# Autodesk Inventor assembly: USE THIS ball intake design
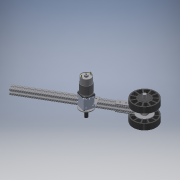
[picture p0: Inventor's stored thumbnail of the model, 180x180]
Saved by Autodesk Inventor 2019 (Build 230136000, 136)
## iProperties
Created: 2019-01-18
Part Number: USE THIS ball intake design
Document SubType Name: Assembly
Designer: s-2513225
Author: s-2513225
## Documents named in this file (9)
- G:\Robotics\Ball Intake 2019\arm assembly left.iam
- G:\Robotics\Ball Intake 2019\wheel tip.ipt
- G:\Robotics\Ball Intake 2019\16in 8020_Shrinkwrap_1.ipt
- G:\Robotics\Ball Intake 2019\0_500_ID_x_1_125_OD_x_0_313_WD_Flanged_Bearing_217-2731.ipt
- G:\Robotics\Ball Intake 2019\motor extension.ipt
- G:\Robotics\Ball Intake 2019\VersaPlanetary_v1_Single_Stage_10_1_with_775_Series.ipt
- G:\Robotics\Ball Intake 2019\am-3480 4IN 500Hex Bore Compliant Wheel.ipt
- G:\Robotics\Ball Intake 2019\hex shaft for wheels.ipt
- G:\Robotics\Ball Intake 2019\wheel spacer.ipt
## Components (12 placed, 8 different names)
1. wheel tip:3 — Mate:14, Mate:34, Flush:9, Flush:10
2. wheel tip:4 — Mate:15, Flush:5, Mate:18, Flush:11
3. 16in 8020_Shrinkwrap_1:1 — Mate:14, Mate:15, Mate:19, Mate:33, Flush:10, Flush:11, Flush:12
4. 0_500_ID_x_1_125_OD_x_0_313_WD_Flanged_Bearing_217-2731:1 — Flush:5, Mate:18, Mate:29
5. 0_500_ID_x_1_125_OD_x_0_313_WD_Flanged_Bearing_217-2731:2 — Mate:34, Flush:9, Mate:35
6. motor extension:1 — Mate:19, Flush:7, Mate:20, Flush:12
7. 0_500_ID_x_1_125_OD_x_0_313_WD_Flanged_Bearing_217-2731:3 — Flush:7, Mate:20, Mate:22, Mate:23
8. VersaPlanetary_v1_Single_Stage_10_1_with_775_Series:1 — Mate:22, Mate:23
9. am-3480 4IN 500Hex Bore Compliant Wheel:1 — Mate:24, Mate:25
10. hex shaft for wheels:1 — Mate:24, Mate:25, Mate:26, Mate:27, Mate:31, Mate:32
11. wheel spacer:1 — Mate:26, Mate:27, Mate:29, Mate:35
12. am-3480 4IN 500Hex Bore Compliant Wheel:2 — Mate:31, Mate:32
## Relationships (23: Mate 17, Flush 6)
- Mate:14: wheel tip:3 ↔ 16in 8020_Shrinkwrap_1:1
- Mate:15: wheel tip:4 ↔ 16in 8020_Shrinkwrap_1:1
- Flush:5: wheel tip:4 ↔ 0_500_ID_x_1_125_OD_x_0_313_WD_Flanged_Bearing_217-2731:1
- Mate:18: wheel tip:4 ↔ 0_500_ID_x_1_125_OD_x_0_313_WD_Flanged_Bearing_217-2731:1
- Mate:19: 16in 8020_Shrinkwrap_1:1 ↔ motor extension:1
- Flush:7: motor extension:1 ↔ 0_500_ID_x_1_125_OD_x_0_313_WD_Flanged_Bearing_217-2731:3
- Mate:20: motor extension:1 ↔ 0_500_ID_x_1_125_OD_x_0_313_WD_Flanged_Bearing_217-2731:3
- Mate:22: 0_500_ID_x_1_125_OD_x_0_313_WD_Flanged_Bearing_217-2731:3 ↔ VersaPlanetary_v1_Single_Stage_10_1_with_775_Series:1
- Mate:23: 0_500_ID_x_1_125_OD_x_0_313_WD_Flanged_Bearing_217-2731:3 ↔ VersaPlanetary_v1_Single_Stage_10_1_with_775_Series:1
- Mate:24: am-3480 4IN 500Hex Bore Compliant Wheel:1 ↔ hex shaft for wheels:1
- Mate:25: am-3480 4IN 500Hex Bore Compliant Wheel:1 ↔ hex shaft for wheels:1
- Mate:26: hex shaft for wheels:1 ↔ wheel spacer:1
- Mate:27: hex shaft for wheels:1 ↔ wheel spacer:1
- Mate:29: 0_500_ID_x_1_125_OD_x_0_313_WD_Flanged_Bearing_217-2731:1 ↔ wheel spacer:1
- Mate:31: hex shaft for wheels:1 ↔ am-3480 4IN 500Hex Bore Compliant Wheel:2
- Mate:32: hex shaft for wheels:1 ↔ am-3480 4IN 500Hex Bore Compliant Wheel:2
- Mate:33: 16in 8020_Shrinkwrap_1:1
- Mate:34: wheel tip:3 ↔ 0_500_ID_x_1_125_OD_x_0_313_WD_Flanged_Bearing_217-2731:2
- Flush:9: wheel tip:3 ↔ 0_500_ID_x_1_125_OD_x_0_313_WD_Flanged_Bearing_217-2731:2
- Mate:35: 0_500_ID_x_1_125_OD_x_0_313_WD_Flanged_Bearing_217-2731:2 ↔ wheel spacer:1
- Flush:10: wheel tip:3 ↔ 16in 8020_Shrinkwrap_1:1
- Flush:11: wheel tip:4 ↔ 16in 8020_Shrinkwrap_1:1
- Flush:12: 16in 8020_Shrinkwrap_1:1 ↔ motor extension:1
